# Autodesk Inventor assembly: Collector Arms v2.0_MIR_MIR_MIR1
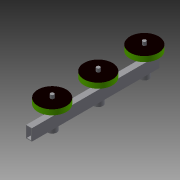
[picture p0: Inventor's stored thumbnail of the model, 180x180]
Saved by Autodesk Inventor 2015 (Build 190159000, 159)
## iProperties
Created: 2015-01-20
Part Number: Collector Arms v2.0_MIR_MIR_MIR1
Document SubType Name: Assembly
Designer: chapale16
Author: chapale16
## Documents named in this file (4)
- \\lhssvr02\Homedirs\Robotics Club\CAD Model 2015\CDR prep\Tote Collector Arms\Collector Arms v2.0_MIR_MIR_MIR1.iam
- \\lhssvr02\Homedirs\Robotics Club\CAD Model 2015\CDR prep\Tote Collector Arms\23.5 in 2 x 1 boxBeam_MIR_MIR_MIR1.ipt
- \\lhssvr02\Homedirs\Robotics Club\CAD Model 2015\CDR prep\Tote Collector Arms\P60 Gear Box_MIR2_MIR_MIR1.ipt
- \\lhssvr02\Homedirs\Robotics Club\CAD Model 2015\CDR prep\Tote Collector Arms\collector arm wheel_MIR2_MIR_MIR1.ipt
## Components (7 placed, 3 different names)
1. 23.5 in 2 x 1 boxBeam_MIR_MIR_MIR1:1 — Flush:9, Mate:1, Flush:1, Flush:3, Mate:5, Flush:5, Mate:8
2. P60 Gear Box_MIR2_MIR_MIR1:1 — Flush:9, Mate:1, Flush:1, Mate:2, Mate:11
3. collector arm wheel_MIR2_MIR_MIR1:1 — Mate:2, Flush:4
4. P60 Gear Box_MIR2_MIR_MIR1:2 — Mate:11, Flush:3, Mate:5, Mate:3, Mate:10
5. collector arm wheel_MIR2_MIR_MIR1:2 — Flush:4, Mate:3, Flush:6
6. P60 Gear Box_MIR2_MIR_MIR1:3 — Mate:10, Flush:5, Mate:8, Mate:6
7. collector arm wheel_MIR2_MIR_MIR1:3 — Flush:6, Mate:6
## Relationships (14: Mate 8, Flush 6)
- Flush:9 (114.3 mm): 23.5 in 2 x 1 boxBeam_MIR_MIR_MIR1:1 ↔ P60 Gear Box_MIR2_MIR_MIR1:1
- Mate:1: 23.5 in 2 x 1 boxBeam_MIR_MIR_MIR1:1 ↔ P60 Gear Box_MIR2_MIR_MIR1:1
- Flush:1: 23.5 in 2 x 1 boxBeam_MIR_MIR_MIR1:1 ↔ P60 Gear Box_MIR2_MIR_MIR1:1
- Mate:2: P60 Gear Box_MIR2_MIR_MIR1:1 ↔ collector arm wheel_MIR2_MIR_MIR1:1
- Mate:11 (161.3154 mm): P60 Gear Box_MIR2_MIR_MIR1:1 ↔ P60 Gear Box_MIR2_MIR_MIR1:2
- Flush:3: 23.5 in 2 x 1 boxBeam_MIR_MIR_MIR1:1 ↔ P60 Gear Box_MIR2_MIR_MIR1:2
- Mate:5: 23.5 in 2 x 1 boxBeam_MIR_MIR_MIR1:1 ↔ P60 Gear Box_MIR2_MIR_MIR1:2
- Flush:4: collector arm wheel_MIR2_MIR_MIR1:1 ↔ collector arm wheel_MIR2_MIR_MIR1:2
- Mate:3: P60 Gear Box_MIR2_MIR_MIR1:2 ↔ collector arm wheel_MIR2_MIR_MIR1:2
- Mate:10 (161.3154 mm): P60 Gear Box_MIR2_MIR_MIR1:2 ↔ P60 Gear Box_MIR2_MIR_MIR1:3
- Flush:5: 23.5 in 2 x 1 boxBeam_MIR_MIR_MIR1:1 ↔ P60 Gear Box_MIR2_MIR_MIR1:3
- Mate:8: 23.5 in 2 x 1 boxBeam_MIR_MIR_MIR1:1 ↔ P60 Gear Box_MIR2_MIR_MIR1:3
- Flush:6: collector arm wheel_MIR2_MIR_MIR1:2 ↔ collector arm wheel_MIR2_MIR_MIR1:3
- Mate:6: P60 Gear Box_MIR2_MIR_MIR1:3 ↔ collector arm wheel_MIR2_MIR_MIR1:3
